# Autodesk Inventor assembly: AstromechV1
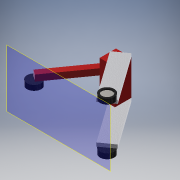
[picture p0: Inventor's stored thumbnail of the model, 180x180]
Saved by Autodesk Inventor 2019 (Build 230136000, 136)
## iProperties
Created: 2020-05-27
Part Number: AstromechV1
Material: Genérico
Document SubType Name: Assembly
Designer: alejo
Author: alejo
## Documents named in this file (3)
- C:\Users\alejo\Documents\UN\RyCSV\Proyecto\CAD\AstromechV1.iam
- C:\Users\alejo\Documents\UN\RyCSV\Proyecto\CAD\structure.ipt
- C:\Users\alejo\Documents\UN\RyCSV\Proyecto\CAD\wheels.ipt
## Components (4 placed, 2 different names)
1. structure:1 — De rotación:1, De rotación:2, De rotación:3
2. wheels:1 — De rotación:3
3. wheels:2 — De rotación:1
4. wheels:3 — De rotación:2
## Relationships (3: RevoluteJoint 3)
- De rotación:1 [RevoluteJoint]: structure:1 ↔ wheels:2
- De rotación:2 [RevoluteJoint]: structure:1 ↔ wheels:3
- De rotación:3 [RevoluteJoint]: structure:1 ↔ wheels:1
